# Autodesk Inventor assembly: YflanecSborka_MIR
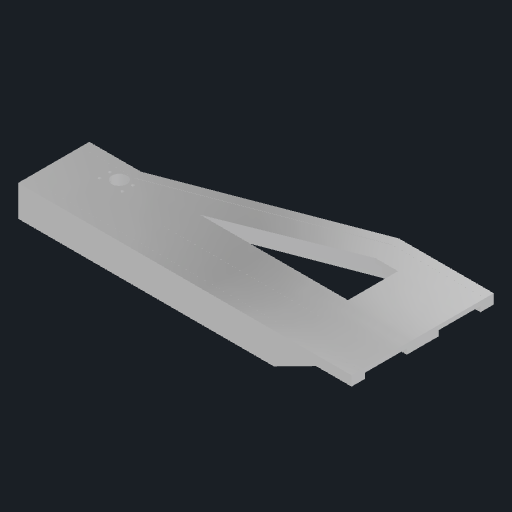
[picture p0: Inventor's stored thumbnail of the model, 512x512]
Saved by Autodesk Inventor 2024 (Build 280153000, 153)
## iProperties
Created: 2023-06-18
Part Number: YflanecSborka_MIR
Document SubType Name: Assembly
Designer: KirikDK
Mass: 15297.3 g
Surface Area: 8753.13 cm^2
Volume: 5665.67 cm^3
Density: 2.7 g/cm^3
Author: KirikDK
## Documents named in this file (5)
- C:\Users\KirikDK\Documents\Stanok2023\YflanecSborka_MIR.iam
- C:\Users\KirikDK\Documents\Stanok2023\YFlanPlate_MIR.ipt
- C:\Users\KirikDK\Documents\Stanok2023\PortalFlanec_MIR.ipt
- C:\Users\KirikDK\Documents\Stanok2023\YflanecYcrepA_MIR.ipt
- C:\Users\KirikDK\Documents\Stanok2023\Y_zigZag_MIR.ipt
## Components (4 placed, 4 different names)
1. YFlanPlate_MIR:1 — Flush:2, Flush:1, Mate:1, Flush:4, Flush:5, Mate:3
2. PortalFlanec_MIR:1 — Flush:2, Flush:1, Mate:1, Flush:3, Mate:2, Flush:6
3. YflanecYcrepA_MIR:1 — Flush:4, Flush:3, Mate:2
4. Y_zigZag_MIR:1 — Flush:6, Flush:5, Mate:3
## Relationships (9: Flush 6, Mate 3)
- Flush:2: YFlanPlate_MIR:1 ↔ PortalFlanec_MIR:1
- Flush:1: YFlanPlate_MIR:1 ↔ PortalFlanec_MIR:1
- Mate:1: YFlanPlate_MIR:1 ↔ PortalFlanec_MIR:1
- Flush:4: YFlanPlate_MIR:1 ↔ YflanecYcrepA_MIR:1
- Flush:3: PortalFlanec_MIR:1 ↔ YflanecYcrepA_MIR:1
- Mate:2: PortalFlanec_MIR:1 ↔ YflanecYcrepA_MIR:1
- Flush:6: PortalFlanec_MIR:1 ↔ Y_zigZag_MIR:1
- Flush:5: YFlanPlate_MIR:1 ↔ Y_zigZag_MIR:1
- Mate:3: YFlanPlate_MIR:1 ↔ Y_zigZag_MIR:1
